# Autodesk Inventor assembly: Panel Top
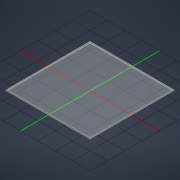
[picture p0: Inventor's stored thumbnail of the model, 180x180]
Saved by Autodesk Inventor 2022.2 (Build 262287010, 287A)
## iProperties
Created: 2022-03-16
Part Number: Panel Top
Document SubType Name: Assembly
Designer: sleib
Author: sleib
## Documents named in this file (3)
- C:\Users\sleib\Projekte\Voron-2\CAD\Inventor\Panel Top.iam
- C:\Users\sleib\Projekte\Voron-2\CAD\Inventor\Panel Top.ipt
- C:\Users\sleib\Projekte\Voron-2\CAD\Inventor\Foamtape Top.ipt
## Components (2 placed, 2 different names)
1. Panel Top:1 — Passend:1, Passend:2, Fluchtend:1
2. Foamtape Top:1 — Passend:1, Passend:2, Fluchtend:1
## Relationships (3: Mate 2, Flush 1)
- Passend:1 [Mate]: Panel Top:1 ↔ Foamtape Top:1
- Passend:2 [Mate]: Panel Top:1 ↔ Foamtape Top:1
- Fluchtend:1 [Flush]: Panel Top:1 ↔ Foamtape Top:1
